# Autodesk Inventor assembly: vp6242_force_sensor_simple_holder
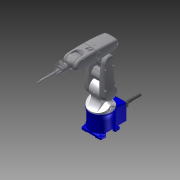
[picture p0: Inventor's stored thumbnail of the model, 180x180]
Saved by Autodesk Inventor 2013 (Build 170138000, 138)
## iProperties
Created: 2013-01-29
Part Number: vp6242_force_sensor_simple_holder
Document SubType Name: Assembly
Designer: Mahisorn
Author: Mahisorn
## Documents named in this file (13)
- E:\mahisorn\documents\hg-ros-pkg\cad\gripper\vp6242_force_sensor_simple_holder.iam
- E:\mahisorn\documents\hg-ros-pkg\cad\gripper\Imported Components\410590-0170-c001_drx\410590-0170-c001_drx.ipt
- E:\mahisorn\documents\hg-ros-pkg\cad\gripper\Imported Components\410590-0170-c002_drx\410590-0170-c002_drx.ipt
- E:\mahisorn\documents\hg-ros-pkg\cad\gripper\Imported Components\410590-0170-c003_drx\410590-0170-c003_drx.ipt
- E:\mahisorn\documents\hg-ros-pkg\cad\gripper\Imported Components\410590-0170-c004_drx\410590-0170-c004_drx.ipt
- E:\mahisorn\documents\hg-ros-pkg\cad\gripper\Imported Components\410590-0170-c005_drx\410590-0170-c005_drx.ipt
- E:\mahisorn\documents\hg-ros-pkg\cad\gripper\Imported Components\410590-0170-c006_drx\410590-0170-c006_drx.ipt
- E:\mahisorn\documents\Inventor\Content Center Files\R2013\en-US\ANSI B18.3.1M(3)\ANSI B18.3.1M - M5x0.8 x 12(5).ipt
- E:\mahisorn\documents\hg-ros-pkg\cad\gripper\plate_cfs055ca501u.ipt
- E:\mahisorn\documents\hg-ros-pkg\cad\gripper\CFS055CA501U.ipt
- E:\mahisorn\documents\hg-ros-pkg\cad\gripper\simple_holder.ipt
- E:\mahisorn\documents\Inventor\Content Center Files\R2013\en-US\ANSI B18.3.1M(5)\ANSI B18.3.1M - M6x1 x 10(3).ipt
- E:\mahisorn\documents\hg-ros-pkg\cad\gripper\pen_pentel_knockle.ipt
## Components (18 placed, 12 different names)
1. Drilled Broached Hexagon Socket Head Cap Screw - 6 Holes - Metric M5x0.8 x 12:2 — Insert:10
2. Drilled Broached Hexagon Socket Head Cap Screw - 6 Holes - Metric M5x0.8 x 12:3 — Insert:8
3. Drilled Broached Hexagon Socket Head Cap Screw - 6 Holes - Metric M5x0.8 x 12:4 — Insert:7
4. Drilled Broached Hexagon Socket Head Cap Screw - 6 Holes - Metric M5x0.8 x 12:5 — Insert:9
5. plate_cfs055ca501u:1 — Insert:6, Insert:7, Insert:8, Insert:9, Insert:10
6. CFS055CA501U:1 — Insert:11
7. simple_holder:1 — Insert:11, Insert:12, Insert:13, Insert:14, Insert:15, Insert:16
8. Drilled Forged Hexagon Socket Head Cap Screw - 6 Holes - Metric M6x1 x 10:1 — Insert:13
9. Drilled Forged Hexagon Socket Head Cap Screw - 6 Holes - Metric M6x1 x 10:2 — Insert:12
10. Drilled Forged Hexagon Socket Head Cap Screw - 6 Holes - Metric M6x1 x 10:3 — Insert:15
11. Drilled Forged Hexagon Socket Head Cap Screw - 6 Holes - Metric M6x1 x 10:4 — Insert:14
12. pen_pentel_knockle:1 — Insert:16
13. 410590-0170-c001_drx:1 — Insert:1
14. 410590-0170-c002_drx:1 — Insert:1, Insert:2
15. 410590-0170-c003_drx:1 — Insert:2, Insert:3
16. 410590-0170-c004_drx:1 — Insert:3, Insert:4
17. 410590-0170-c005_drx:1 — Insert:4, Insert:5
18. 410590-0170-c006_drx:1 — Insert:5, Insert:6
## Relationships (16: Insert 16)
- Insert:1: 410590-0170-c001_drx:1 ↔ 410590-0170-c002_drx:1
- Insert:2: 410590-0170-c002_drx:1 ↔ 410590-0170-c003_drx:1
- Insert:3: 410590-0170-c003_drx:1 ↔ 410590-0170-c004_drx:1
- Insert:4: 410590-0170-c004_drx:1 ↔ 410590-0170-c005_drx:1
- Insert:5: 410590-0170-c005_drx:1 ↔ 410590-0170-c006_drx:1
- Insert:6: plate_cfs055ca501u:1 ↔ 410590-0170-c006_drx:1
- Insert:7: Drilled Broached Hexagon Socket Head Cap Screw - 6 Holes - Metric M5x0.8 x 12:4 ↔ plate_cfs055ca501u:1
- Insert:8: Drilled Broached Hexagon Socket Head Cap Screw - 6 Holes - Metric M5x0.8 x 12:3 ↔ plate_cfs055ca501u:1
- Insert:9: Drilled Broached Hexagon Socket Head Cap Screw - 6 Holes - Metric M5x0.8 x 12:5 ↔ plate_cfs055ca501u:1
- Insert:10: Drilled Broached Hexagon Socket Head Cap Screw - 6 Holes - Metric M5x0.8 x 12:2 ↔ plate_cfs055ca501u:1
- Insert:11: CFS055CA501U:1 ↔ simple_holder:1
- Insert:12: simple_holder:1 ↔ Drilled Forged Hexagon Socket Head Cap Screw - 6 Holes - Metric M6x1 x 10:2
- Insert:13: simple_holder:1 ↔ Drilled Forged Hexagon Socket Head Cap Screw - 6 Holes - Metric M6x1 x 10:1
- Insert:14: simple_holder:1 ↔ Drilled Forged Hexagon Socket Head Cap Screw - 6 Holes - Metric M6x1 x 10:4
- Insert:15: simple_holder:1 ↔ Drilled Forged Hexagon Socket Head Cap Screw - 6 Holes - Metric M6x1 x 10:3
- Insert:16: simple_holder:1 ↔ pen_pentel_knockle:1
